# Autodesk Inventor assembly: Star Piece Proof Assy
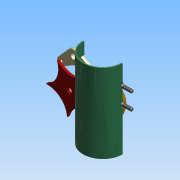
[picture p0: Inventor's stored thumbnail of the model, 180x180]
Saved by Autodesk Inventor 2018.1 (Build 221171000, 171)
## iProperties
Part Number: Star Piece Proof Assy
Document SubType Name: Assembly
Designer: James
Author: James
## Documents named in this file (6)
- C:\Users\admin\Desktop\Ball-Machine\Prototype CAD\Hollow Balls - 40mm_Star Piece New\New Star Piece Proof\Star Piece Proof Assy.iam
- C:\Users\admin\Desktop\Ball-Machine\Prototype CAD\Hollow Balls - 40mm_Star Piece New\Star Piece New.ipt
- C:\Users\admin\Desktop\Ball-Machine\Prototype CAD\Hollow Balls - 40mm_Star Piece New\New Star Piece Proof\Half Cylinder 2.ipt
- C:\Users\admin\Desktop\Ball-Machine\Prototype CAD\Hollow Balls - 40mm_Star Piece New\New Star Piece Proof\Timing_Lever copy.ipt
- C:\Users\admin\Desktop\Ball-Machine\Prototype CAD\Hollow Balls - 40mm_Star Piece New\New Star Piece Proof\Ball 40mm copy.ipt
- C:\Users\admin\Desktop\Ball-Machine\Prototype CAD\Hollow Balls - 40mm_Star Piece New\New Star Piece Proof\Socket Csk Screw - (A2) - M4 x  16.ipt
## Components (6 placed, 5 different names)
1. Star Piece New:1 — Mate:1, Mate:2, Mate:4, Mate:5, Mate:9
2. Half Cylinder 2:1 — Flush:1, Flush:2, Flush:3, Mate:6, Mate:7
3. Timing_Lever copy:1 — Flush:4, Mate:3, Mate:4
4. Ball 40mm copy:1 — Tangent:1, Tangent:2, Mate:9
5. Socket Csk Screw - (A2) - M4 x  16:1 — Mate:6, Flush:5, Mate:8
6. Socket Csk Screw - (A2) - M4 x  16:2 — Mate:7, Flush:5
## Relationships (16: Mate 9, Flush 5, Tangent 2)
- Flush:1: Half Cylinder 2:1
- Flush:2: Half Cylinder 2:1
- Flush:3: Half Cylinder 2:1
- Mate:1 (-38.5 mm): Star Piece New:1
- Mate:2 (1 mm): Star Piece New:1
- Flush:4 (1 mm): Timing_Lever copy:1
- Mate:3 (-38.5 mm): Timing_Lever copy:1
- Mate:4 (35 mm): Star Piece New:1 ↔ Timing_Lever copy:1
- Mate:5 (40 mm): Star Piece New:1
- Mate:6: Half Cylinder 2:1 ↔ Socket Csk Screw - (A2) - M4 x  16:1
- Mate:7: Half Cylinder 2:1 ↔ Socket Csk Screw - (A2) - M4 x  16:2
- Flush:5: Socket Csk Screw - (A2) - M4 x  16:1 ↔ Socket Csk Screw - (A2) - M4 x  16:2
- Mate:8 (21.4 mm): Socket Csk Screw - (A2) - M4 x  16:1
- Tangent:1 (21.4 mm): Ball 40mm copy:1
- Tangent:2 (20 mm): Ball 40mm copy:1
- Mate:9 (20 mm): Star Piece New:1 ↔ Ball 40mm copy:1
